# Autodesk Inventor assembly: gearbox
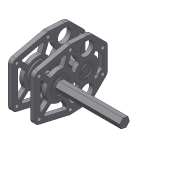
[picture p0: Inventor's stored thumbnail of the model, 180x180]
Saved by Autodesk Inventor 2013 SP1 (Build 170176100, 176)
## iProperties
Created: 2013-11-05
Part Number: gearbox
Document SubType Name: Assembly
Designer: robotics
Author: robotics
## Documents named in this file (7)
- C:\Users\robotics\Documents\GitHub\2014-Preseason-Single-Speed-Gearbox\custom\gearbox.iam
- C:\Users\robotics\Documents\GitHub\2014-Preseason-Single-Speed-Gearbox\custom\BackPlate.ipt
- C:\Users\robotics\Documents\GitHub\2014-Preseason-Single-Speed-Gearbox\custom\LongShaft.ipt
- C:\Users\robotics\Documents\GitHub\2014-Preseason-Single-Speed-Gearbox\custom\RoundBearing-1-2-inch.ipt
- C:\Users\robotics\Documents\GitHub\2014-Preseason-Single-Speed-Gearbox\custom\RoundBearing-3-8-inch.ipt
- C:\Users\robotics\Documents\GitHub\2014-Preseason-Single-Speed-Gearbox\custom\ShortShaft.ipt
- C:\Users\robotics\Documents\GitHub\2014-Preseason-Single-Speed-Gearbox\custom\HexBearing-1-2-inch.ipt
## Components (8 placed, 6 different names)
1. BackPlate:1 — Mate:1, Mate:2, Mate:5, Mate:6
2. LongShaft:1 — Mate:3, Mate:4, Mate:15, Mate:16
3. RoundBearing-1-2-inch:1 — Mate:1, Mate:2, Mate:3, Mate:4
4. RoundBearing-3-8-inch:1 — Mate:5, Mate:6, Mate:7, Mate:8
5. ShortShaft:1 — Mate:7, Mate:8, Mate:9, Mate:10
6. BackPlate:2 — Mate:11, Mate:12, Mate:13, Mate:14
7. RoundBearing-3-8-inch:2 — Mate:9, Mate:10, Mate:13, Mate:14
8. HexBearing-1-2-inch:1 — Mate:11, Mate:12, Mate:15, Mate:16
## Relationships (16: Mate 16)
- Mate:1: BackPlate:1 ↔ RoundBearing-1-2-inch:1
- Mate:2: BackPlate:1 ↔ RoundBearing-1-2-inch:1
- Mate:3: LongShaft:1 ↔ RoundBearing-1-2-inch:1
- Mate:4: LongShaft:1 ↔ RoundBearing-1-2-inch:1
- Mate:5: BackPlate:1 ↔ RoundBearing-3-8-inch:1
- Mate:6: BackPlate:1 ↔ RoundBearing-3-8-inch:1
- Mate:7: RoundBearing-3-8-inch:1 ↔ ShortShaft:1
- Mate:8: RoundBearing-3-8-inch:1 ↔ ShortShaft:1
- Mate:9: ShortShaft:1 ↔ RoundBearing-3-8-inch:2
- Mate:10: ShortShaft:1 ↔ RoundBearing-3-8-inch:2
- Mate:11: BackPlate:2 ↔ HexBearing-1-2-inch:1
- Mate:12: BackPlate:2 ↔ HexBearing-1-2-inch:1
- Mate:13: BackPlate:2 ↔ RoundBearing-3-8-inch:2
- Mate:14: BackPlate:2 ↔ RoundBearing-3-8-inch:2
- Mate:15: LongShaft:1 ↔ HexBearing-1-2-inch:1
- Mate:16: LongShaft:1 ↔ HexBearing-1-2-inch:1
